# Autodesk Inventor assembly: Ensamblaje - Gripper
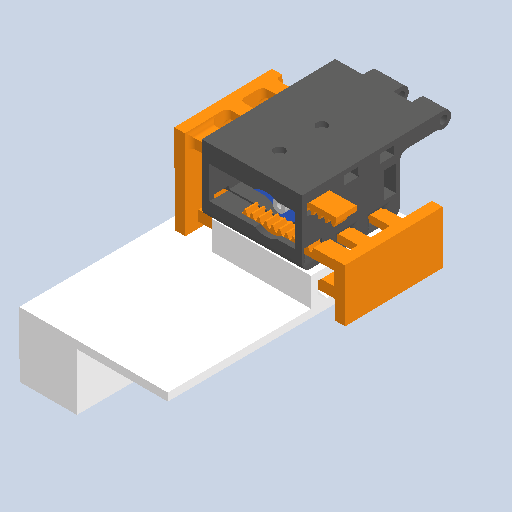
[picture p0: Inventor's stored thumbnail of the model, 512x512]
Saved by Autodesk Inventor 2026 (Build 300175050, 175E)
## iProperties
Created: 2025-10-13
Part Number: Ensamblaje - Gripper
Document SubType Name: Assembly
Designer: bello
Author: bello
## Documents named in this file (6)
- A:\Federico Bellomi\UNLZ\5. Quinto Año\Proyecto Final\Ensamblaje\Gripper\Ensamblaje - Gripper.iam
- A:\Federico Bellomi\UNLZ\5. Quinto Año\Proyecto Final\Ensamblaje\Gripper\Servo SG90\Servo SG90\Servo SG90.ipt
- A:\Federico Bellomi\UNLZ\5. Quinto Año\Proyecto Final\Ensamblaje\Gripper\Base - version 2.ipt
- A:\Federico Bellomi\UNLZ\5. Quinto Año\Proyecto Final\Ensamblaje\Gripper\Pata Izquierda - versión 3.ipt
- A:\Federico Bellomi\UNLZ\5. Quinto Año\Proyecto Final\Ensamblaje\Gripper\Pata derecha - versión 3.ipt
- A:\Federico Bellomi\UNLZ\5. Quinto Año\Proyecto Final\Ensamblaje\Gripper\Base Marcador ECU + Gripper.ipt
## Components (5 placed, 5 different names)
1. Base - version 2:1 — Coincidencia:5, Ángulo:1, Coincidencia:6, Coincidencia:7, Coincidencia:8, Coincidencia:9, Coincidencia:10
2. Servo SG90:1 — Coincidencia:5, Ángulo:1, Coincidencia:6
3. Pata Izquierda - versión 3:1 — Coincidencia:7, Coincidencia:8, Coincidencia:12
4. Pata derecha - versión 3:1 — Coincidencia:9, Coincidencia:10, Coincidencia:11
5. Base Marcador ECU + Gripper:1 — Coincidencia:11, Coincidencia:12
## Relationships (9: Mate 8, Angle 1)
- Coincidencia:5 [Mate]: Base - version 2:1 ↔ Servo SG90:1
- Ángulo:1 [Angle] (180 deg): Base - version 2:1 ↔ Servo SG90:1
- Coincidencia:6 [Mate]: Base - version 2:1 ↔ Servo SG90:1
- Coincidencia:7 [Mate]: Base - version 2:1 ↔ Pata Izquierda - versión 3:1
- Coincidencia:8 [Mate]: Base - version 2:1 ↔ Pata Izquierda - versión 3:1
- Coincidencia:9 [Mate]: Base - version 2:1 ↔ Pata derecha - versión 3:1
- Coincidencia:10 [Mate]: Base - version 2:1 ↔ Pata derecha - versión 3:1
- Coincidencia:11 [Mate]: Pata derecha - versión 3:1 ↔ Base Marcador ECU + Gripper:1
- Coincidencia:12 [Mate]: Pata Izquierda - versión 3:1 ↔ Base Marcador ECU + Gripper:1
